# Autodesk Inventor assembly: ThrustBearing
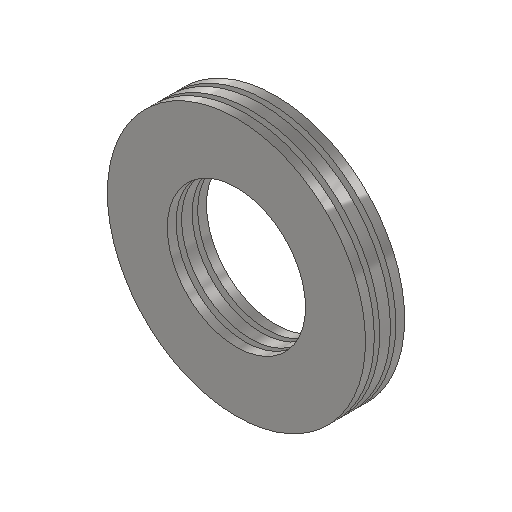
[picture p0: Inventor's stored thumbnail of the model, 512x512]
Saved by Autodesk Inventor 2026.2 (Build 302298000, 298)
## iProperties
Created: 2026-03-25
Part Number: ThrustBearing
Document SubType Name: Assembly
Designer: gaoet
Author: gaoet
## Documents named in this file (3)
- C:\Users\gaoet\OneDrive\Desktop\Scissor 3D Printer\ThrustBearing.iam
- C:\Users\gaoet\OneDrive\Desktop\Scissor 3D Printer\91290A168_Black-Oxide Alloy Steel Socket Head Screw\5909K44_0.032 Thick Washer for 1-2 Shaft Diameter Needle-Roller Thrust Bearing\5909K44_0.032 Thick Washer f.ipt
- C:\Users\gaoet\OneDrive\Desktop\Scissor 3D Printer\91290A168_Black-Oxide Alloy Steel Socket Head Screw\5909K31_Needle-Roller Thrust Bearing\5909K31_Needle-Roller Thrust Bearing.ipt
## Components (3 placed, 2 different names)
1. 5909K44_0.032 Thick Washer f:1 — Mate:2, Mate:3, Mate:4
2. 5909K44_0.032 Thick Washer f:2 — Mate:1, Mate:3
3. 5909K31_Needle-Roller Thrust Bearing:1 — Mate:1, Mate:2, Mate:4
## Relationships (4: Mate 4)
- Mate:1 (0.4961 mm): 5909K44_0.032 Thick Washer f:2 ↔ 5909K31_Needle-Roller Thrust Bearing:1
- Mate:2 (0.4961 mm): 5909K44_0.032 Thick Washer f:1 ↔ 5909K31_Needle-Roller Thrust Bearing:1
- Mate:3: 5909K44_0.032 Thick Washer f:1 ↔ 5909K44_0.032 Thick Washer f:2
- Mate:4: 5909K44_0.032 Thick Washer f:1 ↔ 5909K31_Needle-Roller Thrust Bearing:1
